# Autodesk Inventor assembly: BeamHolder
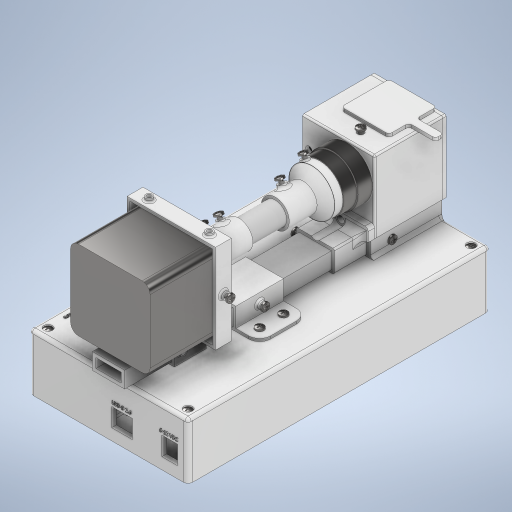
[picture p0: Inventor's stored thumbnail of the model, 512x512]
Saved by Autodesk Inventor 2023 (Build 270158000, 158)
## iProperties
Created: 2022-10-17
Part Number: BeamHolder
Document SubType Name: Assembly
Designer: Miner
Author: Miner
## Documents named in this file (19)
- D:\AKFS\OneDrive - RMIT University\0. Main Research\139. Spectral Camera\01 GitHub\3D Design and Parts\OpenHype assembly.iam
- OpenHype.iam
- D:\AKFS\OneDrive - RMIT University\0. Main Research\139. Spectral Camera\01 GitHub\3D Design and Parts\Source files\Chamber assembly.iam
- D:\AKFS\OneDrive - RMIT University\0. Main Research\139. Spectral Camera\01 GitHub\3D Design and Parts\Source files\Part07 Beam holder on mirror.ipt
- D:\AKFS\OneDrive - RMIT University\0. Main Research\139. Spectral Camera\01 GitHub\3D Design and Parts\Source files\Model Beam.ipt
- D:\AKFS\OneDrive - RMIT University\0. Main Research\139. Spectral Camera\01 GitHub\3D Design and Parts\Source files\Model Camera.ipt
- D:\AKFS\OneDrive - RMIT University\0. Main Research\139. Spectral Camera\01 GitHub\3D Design and Parts\Source files\Part06 Camera holder.ipt
- D:\AKFS\OneDrive - RMIT University\0. Main Research\139. Spectral Camera\01 GitHub\3D Design and Parts\Source files\Model Imaging lens.ipt
- D:\AKFS\OneDrive - RMIT University\0. Main Research\139. Spectral Camera\01 GitHub\3D Design and Parts\Source files\Part04 Imaging lens to spectroscope interface.ipt
- D:\AKFS\OneDrive - RMIT University\0. Main Research\139. Spectral Camera\01 GitHub\3D Design and Parts\Source files\Model Spectroscope.ipt
- D:\AKFS\OneDrive - RMIT University\0. Main Research\139. Spectral Camera\01 GitHub\3D Design and Parts\Source files\Part05 Spectrometer to focusing lens interface.ipt
- D:\AKFS\OneDrive - RMIT University\0. Main Research\139. Spectral Camera\01 GitHub\3D Design and Parts\Source files\Model Camera lens.ipt
- D:\AKFS\OneDrive - RMIT University\0. Main Research\139. Spectral Camera\01 GitHub\3D Design and Parts\Source files\Model Mirro mechanizm.ipt
- C:\Users\Miner\Documents\Inventor\Content Center Files\R2023\en-US\ANSI B18.6.3(05)\ANSI B18.6.3 - 3-56 UNF - 0.1875(17).ipt
- D:\AKFS\OneDrive - RMIT University\0. Main Research\139. Spectral Camera\01 GitHub\3D Design and Parts\Source files\Part08 Beam holder of enclosure.ipt
- D:\AKFS\OneDrive - RMIT University\0. Main Research\139. Spectral Camera\01 GitHub\3D Design and Parts\Source files\Enclosure with Cover.iam
- D:\AKFS\OneDrive - RMIT University\0. Main Research\139. Spectral Camera\01 GitHub\3D Design and Parts\Source files\Model Voltemeter.ipt
- D:\AKFS\OneDrive - RMIT University\0. Main Research\139. Spectral Camera\01 GitHub\3D Design and Parts\Source files\Model Mirrorcontroller heatsink.ipt
- D:\AKFS\OneDrive - RMIT University\0. Main Research\139. Spectral Camera\01 GitHub\3D Design and Parts\Source files\Part03 Dust cover.ipt
## Components (38 placed, 17 different names)
1. MirrorRoom [sub-assembly] — Flush:1, Rigid:2, Rigid:4, Rotational:13, Rigid:5, Flush:3, Mate:10, Mate:11
2. Enclosure with Cover:1 [sub-assembly] — Mate:5, Mate:6, Flush:3, Flush:4, Mate:7, Mate:8, Mate:9, Rigid:8, Rotational:20, Rotational:21, Rotational:22, Rotational:24, Rotational:25, Rotational:26, Rotational:27
3. Part04 Imaging lens to spectroscope interface:1 — Rotational:1, Rigid:3, Rotational:4, Rotational:5
4. Part03 Dust cover:1 — Mate:10, Mate:11
5. Part05 Spectrometer to focusing lens interface:1 — Rotational:2, Rotational:3, Rotational:6, Rotational:7
6. Part06 Camera holder:1 — Rigid:1, Rigid:7, Rotational:14, Mate:12, Mate:13
7. Part07 Beam holder on mirror:1 — Flush:1, Flush:2, Rotational:8, Rigid:5
8. Part08 Beam holder of enclosure:1 — Mate:3, Mate:4, Rotational:16, Rotational:17, Rotational:18, Rotational:19, Rotational:23
9. Model Beam:1 — Flush:2, Mate:3, Mate:4, Mate:5, Mate:6, Mate:12, Mate:13
10. Model Camera:1 — Rigid:1
11. Model Imaging lens:1 — Rigid:2, Rotational:1
12. Model Spectroscope:1 — Rigid:3, Rotational:2
13. Model Camera lens:1 — Rotational:3
14. Model Voltemeter:1 — Flush:4, Mate:7
15. Model Mirrorcontroller heatsink:1 — Mate:8, Mate:9
16. Model Mirro mechanizm:1 — Rigid:4, Mate:1, Mate:2
17. Cross Recessed Binding Head Machine Screw - Type II - Inch No. 3 - 56 - 3/16:1 — Rotational:4
18. Cross Recessed Binding Head Machine Screw - Type II - Inch No. 3 - 56 - 3/16:2 — Rotational:7
19. Cross Recessed Binding Head Machine Screw - Type II - Inch No. 3 - 56 - 3/16:3 — Rotational:6
20. Cross Recessed Binding Head Machine Screw - Type II - Inch No. 3 - 56 - 3/16:5 — Rigid:7
21. Cross Recessed Binding Head Machine Screw - Type II - Inch No. 3 - 56 - 3/16:6 — Rotational:8
22. Cross Recessed Binding Head Machine Screw - Type II - Inch No. 3 - 56 - 3/16:7 — Rotational:5
23. Cross Recessed Binding Head Machine Screw - Type II - Inch No. 3 - 56 - 3/16:11 — Rotational:13
24. Cross Recessed Binding Head Machine Screw - Type II - Inch No. 3 - 56 - 3/16:12 — Rotational:14
25. Cross Recessed Binding Head Machine Screw - Type II - Inch No. 3 - 56 - 3/16:13
26. Cross Recessed Binding Head Machine Screw - Type II - Inch No. 3 - 56 - 3/16:14 — Rotational:16
27. Cross Recessed Binding Head Machine Screw - Type II - Inch No. 3 - 56 - 3/16:15 — Rotational:17
28. Cross Recessed Binding Head Machine Screw - Type II - Inch No. 3 - 56 - 3/16:16 — Rotational:18
29. Cross Recessed Binding Head Machine Screw - Type II - Inch No. 3 - 56 - 3/16:17 — Rotational:19
30. Cross Recessed Binding Head Machine Screw - Type II - Inch No. 3 - 56 - 3/16:18 — Rigid:8
31. Cross Recessed Binding Head Machine Screw - Type II - Inch No. 3 - 56 - 3/16:19 — Rotational:21
32. Cross Recessed Binding Head Machine Screw - Type II - Inch No. 3 - 56 - 3/16:20 — Rotational:22
33. Cross Recessed Binding Head Machine Screw - Type II - Inch No. 3 - 56 - 3/16:21 — Rotational:20
34. Cross Recessed Binding Head Machine Screw - Type II - Inch No. 3 - 56 - 3/16:22 — Rotational:23
35. Cross Recessed Binding Head Machine Screw - Type II - Inch No. 3 - 56 - 3/16:23 — Rotational:24
36. Cross Recessed Binding Head Machine Screw - Type II - Inch No. 3 - 56 - 3/16:24 — Rotational:25
37. Cross Recessed Binding Head Machine Screw - Type II - Inch No. 3 - 56 - 3/16:25 — Rotational:26
38. Cross Recessed Binding Head Machine Screw - Type II - Inch No. 3 - 56 - 3/16:26 — Rotational:27
## Relationships (46: RevoluteJoint 22, Mate 13, WeldJoint 7, Flush 4)
- Flush:1: MirrorRoom ↔ Part07 Beam holder on mirror:1
- Flush:2: Part07 Beam holder on mirror:1 ↔ Model Beam:1
- Rigid:1 [WeldJoint] (1.8 mm): Part06 Camera holder:1 ↔ Model Camera:1
- Rigid:2 [WeldJoint]: MirrorRoom ↔ Model Imaging lens:1
- Rotational:1 [RevoluteJoint]: Part04 Imaging lens to spectroscope interface:1 ↔ Model Imaging lens:1
- Rigid:3 [WeldJoint]: Part04 Imaging lens to spectroscope interface:1 ↔ Model Spectroscope:1
- Rotational:2 [RevoluteJoint]: Part05 Spectrometer to focusing lens interface:1 ↔ Model Spectroscope:1
- Rotational:3 [RevoluteJoint]: Part05 Spectrometer to focusing lens interface:1 ↔ Model Camera lens:1
- Rigid:4 [WeldJoint]: MirrorRoom ↔ Model Mirro mechanizm:1
- Rotational:4 [RevoluteJoint] (-2 mm): Part04 Imaging lens to spectroscope interface:1 ↔ Cross Recessed Binding Head Machine Screw - Type II - Inch No. 3 - 56 - 3/16:1
- Rotational:5 [RevoluteJoint] (-2 mm): Part04 Imaging lens to spectroscope interface:1 ↔ Cross Recessed Binding Head Machine Screw - Type II - Inch No. 3 - 56 - 3/16:7
- Rotational:6 [RevoluteJoint] (-2 mm): Part05 Spectrometer to focusing lens interface:1 ↔ Cross Recessed Binding Head Machine Screw - Type II - Inch No. 3 - 56 - 3/16:3
- Rotational:7 [RevoluteJoint] (-2 mm): Part05 Spectrometer to focusing lens interface:1 ↔ Cross Recessed Binding Head Machine Screw - Type II - Inch No. 3 - 56 - 3/16:2
- Rotational:8 [RevoluteJoint] (-2 mm): Part07 Beam holder on mirror:1 ↔ Cross Recessed Binding Head Machine Screw - Type II - Inch No. 3 - 56 - 3/16:6
- Rotational:13 [RevoluteJoint] (-2 mm): MirrorRoom ↔ Cross Recessed Binding Head Machine Screw - Type II - Inch No. 3 - 56 - 3/16:11
- Mate:1: Model Mirro mechanizm:1
- Mate:2: Model Mirro mechanizm:1
- Rigid:5 [WeldJoint]: MirrorRoom ↔ Part07 Beam holder on mirror:1
- Rigid:7 [WeldJoint] (2 mm): Part06 Camera holder:1 ↔ Cross Recessed Binding Head Machine Screw - Type II - Inch No. 3 - 56 - 3/16:5
- Rotational:14 [RevoluteJoint] (2 mm): Part06 Camera holder:1 ↔ Cross Recessed Binding Head Machine Screw - Type II - Inch No. 3 - 56 - 3/16:12
- Mate:3: Part08 Beam holder of enclosure:1 ↔ Model Beam:1
- Mate:4: Part08 Beam holder of enclosure:1 ↔ Model Beam:1
- Rotational:16 [RevoluteJoint]: Part08 Beam holder of enclosure:1 ↔ Cross Recessed Binding Head Machine Screw - Type II - Inch No. 3 - 56 - 3/16:14
- Rotational:17 [RevoluteJoint]: Part08 Beam holder of enclosure:1 ↔ Cross Recessed Binding Head Machine Screw - Type II - Inch No. 3 - 56 - 3/16:15
- Rotational:18 [RevoluteJoint]: Part08 Beam holder of enclosure:1 ↔ Cross Recessed Binding Head Machine Screw - Type II - Inch No. 3 - 56 - 3/16:16
- Rotational:19 [RevoluteJoint]: Part08 Beam holder of enclosure:1 ↔ Cross Recessed Binding Head Machine Screw - Type II - Inch No. 3 - 56 - 3/16:17
- Mate:5: Enclosure with Cover:1 ↔ Model Beam:1
- Mate:6: Enclosure with Cover:1 ↔ Model Beam:1
- Flush:3: MirrorRoom ↔ Enclosure with Cover:1
- Flush:4: Enclosure with Cover:1 ↔ Model Voltemeter:1
- Mate:7: Enclosure with Cover:1 ↔ Model Voltemeter:1
- Mate:8: Enclosure with Cover:1 ↔ Model Mirrorcontroller heatsink:1
- Mate:9: Enclosure with Cover:1 ↔ Model Mirrorcontroller heatsink:1
- Rigid:8 [WeldJoint]: Enclosure with Cover:1 ↔ Cross Recessed Binding Head Machine Screw - Type II - Inch No. 3 - 56 - 3/16:18
- Rotational:20 [RevoluteJoint]: Enclosure with Cover:1 ↔ Cross Recessed Binding Head Machine Screw - Type II - Inch No. 3 - 56 - 3/16:21
- Rotational:21 [RevoluteJoint]: Enclosure with Cover:1 ↔ Cross Recessed Binding Head Machine Screw - Type II - Inch No. 3 - 56 - 3/16:19
- Rotational:22 [RevoluteJoint]: Enclosure with Cover:1 ↔ Cross Recessed Binding Head Machine Screw - Type II - Inch No. 3 - 56 - 3/16:20
- Rotational:23 [RevoluteJoint] (-1 mm): Part08 Beam holder of enclosure:1 ↔ Cross Recessed Binding Head Machine Screw - Type II - Inch No. 3 - 56 - 3/16:22
- Rotational:24 [RevoluteJoint] (-1 mm): Enclosure with Cover:1 ↔ Cross Recessed Binding Head Machine Screw - Type II - Inch No. 3 - 56 - 3/16:23
- Rotational:25 [RevoluteJoint] (-1 mm): Enclosure with Cover:1 ↔ Cross Recessed Binding Head Machine Screw - Type II - Inch No. 3 - 56 - 3/16:24
- Rotational:26 [RevoluteJoint] (3 mm): Enclosure with Cover:1 ↔ Cross Recessed Binding Head Machine Screw - Type II - Inch No. 3 - 56 - 3/16:25
- Rotational:27 [RevoluteJoint] (3 mm): Enclosure with Cover:1 ↔ Cross Recessed Binding Head Machine Screw - Type II - Inch No. 3 - 56 - 3/16:26
- Mate:10: MirrorRoom ↔ Part03 Dust cover:1
- Mate:11: MirrorRoom ↔ Part03 Dust cover:1
- Mate:12: Part06 Camera holder:1 ↔ Model Beam:1
- Mate:13: Part06 Camera holder:1 ↔ Model Beam:1
